# Autodesk Inventor assembly: assembled servo block attempt to fix
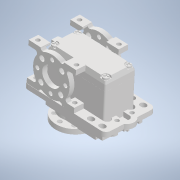
[picture p0: Inventor's stored thumbnail of the model, 180x180]
Saved by Autodesk Inventor 2021 (Build 250183000, 183)
## iProperties
Created: 2020-09-23
Part Number: assembled servo block attempt to fix
Document SubType Name: Assembly
Designer: elois
Author: elois
## Documents named in this file (5)
- C:\Users\Owner\Documents\GitHub\CAD-2021-Ultimate_Goal\Wobble Goal\assembled servo block attempt to fix.iam
- C:\Users\Owner\Documents\GitHub\CAD-2021-Ultimate_Goal\ServoCity\servo mount.ipt
- C:\Users\Owner\Documents\GitHub\CAD-2021-Ultimate_Goal\ServoCity\servo side brackets.ipt
- C:\Users\Owner\Documents\GitHub\CAD-2021-Ultimate_Goal\ServoCity\go builda servo(speed).ipt
- C:\Users\Owner\Documents\GitHub\CAD-2021-Ultimate_Goal\ServoCity\525125_MIR.ipt
## Components (5 placed, 4 different names)
1. servo mount:1 — Mate:22, Mate:23, Mate:24, Mate:25, Mate:26, Mate:27
2. servo side brackets:1 — Mate:23, Mate:26
3. go builda servo(speed):1 — Mate:24, Mate:25, Mate:28, Mate:29
4. 525125_MIR:1 — Mate:28, Mate:29
5. servo side brackets:2 — Mate:22, Mate:27
## Relationships (8: Mate 8)
- Mate:22: servo mount:1 ↔ servo side brackets:2
- Mate:23: servo mount:1 ↔ servo side brackets:1
- Mate:24: servo mount:1 ↔ go builda servo(speed):1
- Mate:25: servo mount:1 ↔ go builda servo(speed):1
- Mate:26: servo mount:1 ↔ servo side brackets:1
- Mate:27: servo mount:1 ↔ servo side brackets:2
- Mate:28: go builda servo(speed):1 ↔ 525125_MIR:1
- Mate:29: go builda servo(speed):1 ↔ 525125_MIR:1
